# Autodesk Inventor assembly: Square Rounded Caps
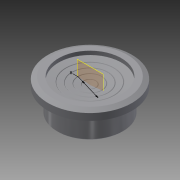
[picture p0: Inventor's stored thumbnail of the model, 180x180]
Saved by Autodesk Inventor 2018 (Build 220112000, 112)
## iProperties
Created: 2017-12-12
Part Number: Square Rounded Caps
Document SubType Name: Assembly
Designer: Rus
Author: Rus
## Documents named in this file (3)
- E:\Libraries\Documents\3D Models\Spinners and Tops\Caps 8mm\Square Rounded Caps\Square Rounded Caps.iam
- E:\Libraries\Documents\3D Models\Spinners and Tops\Caps 8mm\Square Rounded Caps\Caps 8mm Square Rounded Caps Male.ipt
- E:\Libraries\Documents\3D Models\Spinners and Tops\Caps 8mm\Square Rounded Caps\608-bearing.ipt
## Components (2 placed, 2 different names)
1. Caps 8mm Square Rounded Caps Male:1 — Insert:1
2. 608-bearing:1 — Insert:1
## Relationships (1: Insert 1)
- Insert:1: Caps 8mm Square Rounded Caps Male:1 ↔ 608-bearing:1
